# Autodesk Inventor assembly: AASTRC Middle case cover assembly
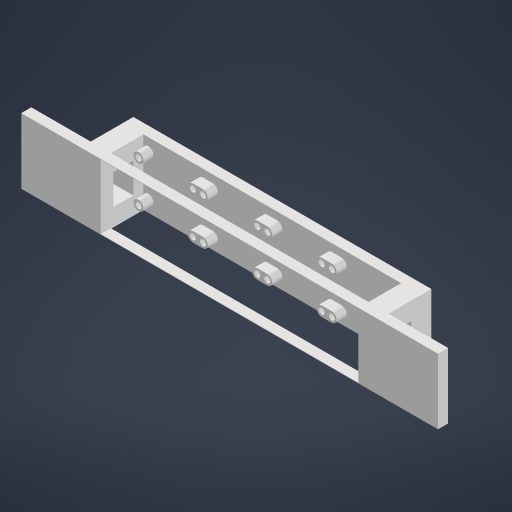
[picture p0: Inventor's stored thumbnail of the model, 512x512]
Saved by Autodesk Inventor 2024.2 (Build 282272000, 272)
## iProperties
Created: 2023-07-17
Part Number: AASTRC Middle case cover assembly
Document SubType Name: Assembly
Designer: wodyd
Author: wodyd
## Documents named in this file (4)
- C:\Users\6gioc\OneDrive\AAST\PART\AAST Remote Controler\AASTRC Middle case cover assembly.iam
- C:\Users\6gioc\OneDrive\AAST\PART\AAST Remote Controler\AASTRC Middle case cover.ipt
- C:\Users\6gioc\OneDrive\AAST\PART\AAST Remote Controler\dot matrix 4.ipt
- C:\Users\6gioc\OneDrive\AAST\PART\AAST Remote Controler\dot matrix cover.ipt
## Components (3 placed, 3 different names)
1. AASTRC Middle case cover:1 — 강체:1, 플러쉬:1, 강체:2
2. dot matrix 4:1 — 강체:1
3. dot matrix cover:1 — 플러쉬:1, 강체:2
## Relationships (3: WeldJoint 2, Flush 1)
- 강체:1 [WeldJoint]: AASTRC Middle case cover:1 ↔ dot matrix 4:1
- 플러쉬:1 [Flush]: AASTRC Middle case cover:1 ↔ dot matrix cover:1
- 강체:2 [WeldJoint]: AASTRC Middle case cover:1 ↔ dot matrix cover:1
